# Autodesk Inventor assembly: Lower Static Arms
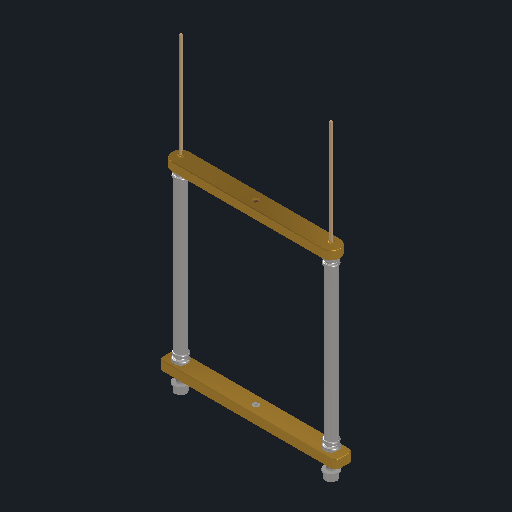
[picture p0: Inventor's stored thumbnail of the model, 512x512]
Saved by Autodesk Inventor 2027.1 (Build 311270010, 270A)
## iProperties
Created: 2025-09-16
Document SubType Name: Assembly
Designer: SD
Mass: 1267.89 g
Surface Area: 532.298 cm^2
Volume: 153.651 cm^3
Density: 8.25173 g/cm^3
Project: Automatic Tea Steeping mechanism
Part Number: Lower Static Arms
BOM-Mass: 1.26789
BOM-Area: 0.053
Author: SD
Title: Lower Static Arms
## Documents named in this file (10)
- C:\Users\Gamer\Documents\Projects\Auto Tea Steeper\Public Version\Automatic Tea Steeper\CAD\Workspace\Lower Static Arms.iam
- C:\Users\Gamer\Documents\Projects\Auto Tea Steeper\Public Version\Automatic Tea Steeper\CAD\Workspace\Lower Arm Brass Plate.ipt
- C:\Users\Gamer\Documents\Projects\Auto Tea Steeper\Public Version\Automatic Tea Steeper\CAD\Workspace\Lower Arm Brass Plate - 2.ipt
- C:\Users\Gamer\Documents\Projects\Auto Tea Steeper\Public Version\Automatic Tea Steeper\CAD\Workspace\Ball Bearing-1.ipt
- C:\Users\Gamer\Documents\Projects\Auto Tea Steeper\Public Version\Automatic Tea Steeper\CAD\Workspace\Domed End Rod 150mm.ipt
- C:\Users\Gamer\Documents\Projects\Auto Tea Steeper\Public Version\Automatic Tea Steeper\CAD\Workspace\Hardware\Allen Key 8x40mm.ipt
- C:\Users\Gamer\Documents\Projects\Auto Tea Steeper\Public Version\Automatic Tea Steeper\CAD\Workspace\Hardware\Brass M3 Hex Nut.ipt
- C:\Users\Gamer\Documents\Projects\Auto Tea Steeper\Public Version\Automatic Tea Steeper\CAD\Workspace\Hardware\8mm Washer.ipt
- C:\Users\Gamer\Documents\Projects\Auto Tea Steeper\Public Version\Automatic Tea Steeper\CAD\Workspace\Lower Arm Support.ipt
- C:\Users\Gamer\Documents\Projects\Auto Tea Steeper\Public Version\Automatic Tea Steeper\CAD\Workspace\FM-306-10.ipt
## Components (14 placed, 9 different names)
1. Lower Arm Brass Plate:1 — Mate:7, Mate:8, Mate:14, Mate:15, Mate:16, Mate:27, Mate:32
2. Lower Arm Brass Plate - 2:1 — Mate:1, Mate:2, Flush:14, Mate:20, Mate:21, Mate:28, Mate:29, Mate:30, Mate:33, Mate:34
3. 683ZZ Ball Bearing:1 — Mate:7, Mate:8
4. Domed End Rod 150mm:1 — Flush:14, Flush:15, Mate:18, Mate:34
5. Domed End Rod 150mm:2 — Flush:15, Mate:19, Mate:30
6. FM-306-10:1 — Mate:1, Mate:2
7. Allen Key 8x40mm:1 — Mate:14, Mate:15, Flush:16, Mate:22, Mate:23, Mate:31
8. Allen Key 8x40mm:2 — Mate:16, Flush:16, Mate:24, Mate:25, Mate:26
9. Brass M3 Hex Nut:1 — Mate:19, Mate:20
10. Brass M3 Hex Nut:2 — Mate:18, Mate:21
11. ISO 7089 8:1 — Mate:22, Mate:23
12. ISO 7089 8:2 — Mate:24, Mate:25
13. Lower Arm Support:1 — Mate:26, Mate:27, Mate:28, Mate:29
14. Lower Arm Support:2 — Mate:31, Mate:32, Mate:33
## Relationships (27: Mate 24, Flush 3)
- Mate:1: Lower Arm Brass Plate - 2:1 ↔ FM-306-10:1
- Mate:2: Lower Arm Brass Plate - 2:1 ↔ FM-306-10:1
- Mate:7: Lower Arm Brass Plate:1 ↔ 683ZZ Ball Bearing:1
- Mate:8: Lower Arm Brass Plate:1 ↔ 683ZZ Ball Bearing:1
- Flush:14 (120 mm): Lower Arm Brass Plate - 2:1 ↔ Domed End Rod 150mm:1
- Flush:15: Domed End Rod 150mm:1 ↔ Domed End Rod 150mm:2
- Mate:14: Lower Arm Brass Plate:1 ↔ Allen Key 8x40mm:1
- Mate:15 (11.5 mm): Lower Arm Brass Plate:1 ↔ Allen Key 8x40mm:1
- Mate:16: Lower Arm Brass Plate:1 ↔ Allen Key 8x40mm:2
- Mate:18: Domed End Rod 150mm:1 ↔ Brass M3 Hex Nut:2
- Mate:19: Domed End Rod 150mm:2 ↔ Brass M3 Hex Nut:1
- Mate:20: Lower Arm Brass Plate - 2:1 ↔ Brass M3 Hex Nut:1
- Mate:21: Lower Arm Brass Plate - 2:1 ↔ Brass M3 Hex Nut:2
- Flush:16: Allen Key 8x40mm:1 ↔ Allen Key 8x40mm:2
- Mate:22: Allen Key 8x40mm:1 ↔ ISO 7089 8:1
- Mate:23: Allen Key 8x40mm:1 ↔ ISO 7089 8:1
- Mate:24: Allen Key 8x40mm:2 ↔ ISO 7089 8:2
- Mate:25: Allen Key 8x40mm:2 ↔ ISO 7089 8:2
- Mate:26: Allen Key 8x40mm:2 ↔ Lower Arm Support:1
- Mate:27: Lower Arm Brass Plate:1 ↔ Lower Arm Support:1
- Mate:28: Lower Arm Brass Plate - 2:1 ↔ Lower Arm Support:1
- Mate:29: Lower Arm Brass Plate - 2:1 ↔ Lower Arm Support:1
- Mate:30: Lower Arm Brass Plate - 2:1 ↔ Domed End Rod 150mm:2
- Mate:31: Allen Key 8x40mm:1 ↔ Lower Arm Support:2
- Mate:32: Lower Arm Brass Plate:1 ↔ Lower Arm Support:2
- Mate:33: Lower Arm Brass Plate - 2:1 ↔ Lower Arm Support:2
- Mate:34: Lower Arm Brass Plate - 2:1 ↔ Domed End Rod 150mm:1
